# Autodesk Inventor assembly: LZM-15ZT flowmeter
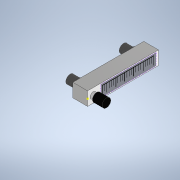
[picture p0: Inventor's stored thumbnail of the model, 180x180]
Saved by Autodesk Inventor 2020.3 (Build 243373000, 373)
## iProperties
Created: 2020-08-06
Part Number: LZM-15ZT flowmeter
Document SubType Name: Assembly
Designer: Bruno
Author: Bruno
## Documents named in this file (5)
- C:\Users\Bruno\Desktop\Rotameter\LZM-15ZT flowmeter.iam
- C:\Users\Bruno\Desktop\Rotameter\LZM-15ZT flowmeter parts\LZM-15ZT_rotameter_06-6_M3-H.ipt
- C:\Users\Bruno\Desktop\Rotameter\LZM-15ZT flowmeter parts\din m6-10 Flat point socket set screw.ipt
- C:\Users\Bruno\Desktop\Rotameter\LZM-15ZT flowmeter parts\din_6902-a_m6-200hv.ipt
- C:\Users\Bruno\Desktop\Rotameter\LZM-15ZT flowmeter parts\nut_din934_m6-10.ipt
## Components (7 placed, 4 different names)
1. LZM-15ZT_rotameter_06-6_M3-H:1 — Cylindrical:1, Cylindrical:2, Cylindrical:3, Cylindrical:4
2. din m6-10 Flat point socket set screw:1 — Cylindrical:1
3. din m6-10 Flat point socket set screw:2 — Cylindrical:2
4. din_6902-a_m6-200hv:1 — Cylindrical:4, Rotational:1
5. din_6902-a_m6-200hv:2 — Cylindrical:3, Cylindrical:5
6. nut_din934_m6-10:1 — Cylindrical:5
7. nut_din934_m6-10:2 — Rotational:1
## Relationships (6: CylindricalJoint 5, RevoluteJoint 1)
- Cylindrical:1: LZM-15ZT_rotameter_06-6_M3-H:1 ↔ din m6-10 Flat point socket set screw:1
- Cylindrical:2: LZM-15ZT_rotameter_06-6_M3-H:1 ↔ din m6-10 Flat point socket set screw:2
- Cylindrical:3: LZM-15ZT_rotameter_06-6_M3-H:1 ↔ din_6902-a_m6-200hv:2
- Cylindrical:4: LZM-15ZT_rotameter_06-6_M3-H:1 ↔ din_6902-a_m6-200hv:1
- Cylindrical:5: din_6902-a_m6-200hv:2 ↔ nut_din934_m6-10:1
- Rotational:1 [RevoluteJoint] (1 mm): din_6902-a_m6-200hv:1 ↔ nut_din934_m6-10:2
